# Autodesk Inventor assembly: Headlight
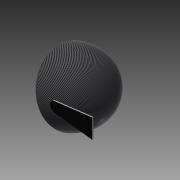
[picture p0: Inventor's stored thumbnail of the model, 180x180]
Saved by Autodesk Inventor 2016 (Build 200138000, 138)
## iProperties
Created: 2015-08-08
Part Number: Headlight
Document SubType Name: Assembly
Designer: Yann
Author: Yann
## Documents named in this file (3)
- C:\Users\Yann\Documents\GitHub\Bikair_CAD\Source\Front_Train\Headlight.iam
- C:\Users\Yann\Documents\GitHub\Bikair_CAD\Source\Front_Train\Headlight\Headlight_Round_Body.ipt
- C:\Users\Yann\Documents\GitHub\Bikair_CAD\Source\Front_Train\Headlight\Headlight_Mounting_Bracket.ipt
## Components (2 placed, 2 different names)
1. Headlight_Round_Body:1 — Flush:5
2. Headlight_Mounting_Bracket:1
## Relationships (1: Flush 1)
- Flush:5: Headlight_Round_Body:1
